# Autodesk Inventor assembly: Assembly
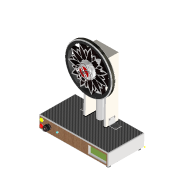
[picture p0: Inventor's stored thumbnail of the model, 180x180]
Saved by Autodesk Inventor 2021 (Build 250183000, 183)
## iProperties
Created: 2021-06-24
Part Number: Assembly
Document SubType Name: Assembly
Designer: RahulRC
Author: RahulRC
## Documents named in this file (10)
- C:\Users\RahulRC\Desktop\Assignments\Exploration\Course_Project\3DModeling\Assembly\Assembly.iam
- C:\Users\RahulRC\Desktop\Assignments\Exploration\Course_Project\3DModeling\Assembly\Design.ipt
- C:\Users\RahulRC\Desktop\Assignments\Exploration\Course_Project\3DModeling\Assembly\DCMotorv2.ipt
- C:\Users\RahulRC\Desktop\Assignments\Exploration\Course_Project\3DModeling\Assembly\rod 2 (1).ipt
- C:\Users\RahulRC\Desktop\Assignments\Exploration\Course_Project\3DModeling\Assembly\buzzer.ipt
- C:\Users\RahulRC\Desktop\Assignments\Exploration\Course_Project\3DModeling\Assembly\base 2.ipt
- C:\Users\RahulRC\Desktop\Assignments\Exploration\Course_Project\3DModeling\Assembly\Attaching Component.ipt
- C:\Users\RahulRC\Desktop\Assignments\Exploration\Course_Project\3DModeling\Assembly\Clamps.ipt
- C:\Users\RahulRC\Desktop\Assignments\Exploration\Course_Project\3DModeling\Assembly\Bolt.ipt
- C:\Users\RahulRC\Desktop\Assignments\Exploration\Course_Project\3DModeling\Assembly\Bolt2.ipt
## Components (17 placed, 9 different names)
1. Design:1 — Mate:1, Mate:2, Angle:1
2. DCMotorv2:1 — Mate:1, Mate:2, Mate:6, Mate:7, Mate:8, Angle:1
3. rod 2 (1):1 — Mate:3, Mate:5
4. buzzer:1 — Mate:4
5. base 2:1 — Mate:3, Mate:4, Mate:9, Mate:10, Mate:21, Mate:22
6. Attaching Component:1 — Mate:5, Mate:6, Mate:7, Mate:8, Mate:31, Mate:32
7. Clamps:1 — Mate:9, Mate:10, Mate:13, Mate:14, Mate:15, Mate:16, Mate:17, Mate:18, Mate:19, Mate:20
8. Bolt:1 — Mate:13, Mate:14
9. Bolt:2 — Mate:17, Mate:19
10. Bolt:3 — Mate:15, Mate:16
11. Bolt:4 — Mate:18, Mate:20
12. Clamps:2 — Mate:21, Mate:22, Mate:23, Mate:24, Mate:25, Mate:26, Mate:27, Mate:28, Mate:29, Mate:30
13. Bolt:5 — Mate:26, Mate:27
14. Bolt:6 — Mate:24, Mate:29
15. Bolt:7 — Mate:25, Mate:28
16. Bolt:8 — Mate:23, Mate:30
17. Bolt2:1 — Mate:31, Mate:32
## Relationships (31: Mate 30, Angle 1)
- Mate:1: Design:1 ↔ DCMotorv2:1
- Mate:2 (2.54 mm): Design:1 ↔ DCMotorv2:1
- Mate:3 (-1 mm): rod 2 (1):1 ↔ base 2:1
- Mate:4: buzzer:1 ↔ base 2:1
- Mate:5: rod 2 (1):1 ↔ Attaching Component:1
- Mate:6: DCMotorv2:1 ↔ Attaching Component:1
- Mate:7: DCMotorv2:1 ↔ Attaching Component:1
- Mate:8: DCMotorv2:1 ↔ Attaching Component:1
- Angle:1 (99640 deg): Design:1 ↔ DCMotorv2:1
- Mate:9: base 2:1 ↔ Clamps:1
- Mate:10: base 2:1 ↔ Clamps:1
- Mate:13: Clamps:1 ↔ Bolt:1
- Mate:14: Clamps:1 ↔ Bolt:1
- Mate:15: Clamps:1 ↔ Bolt:3
- Mate:16: Clamps:1 ↔ Bolt:3
- Mate:17: Clamps:1 ↔ Bolt:2
- Mate:18: Clamps:1 ↔ Bolt:4
- Mate:19: Clamps:1 ↔ Bolt:2
- Mate:20: Clamps:1 ↔ Bolt:4
- Mate:21: base 2:1 ↔ Clamps:2
- Mate:22: base 2:1 ↔ Clamps:2
- Mate:23: Clamps:2 ↔ Bolt:8
- Mate:24: Clamps:2 ↔ Bolt:6
- Mate:25: Clamps:2 ↔ Bolt:7
- Mate:26: Clamps:2 ↔ Bolt:5
- Mate:27: Clamps:2 ↔ Bolt:5
- Mate:28: Clamps:2 ↔ Bolt:7
- Mate:29: Clamps:2 ↔ Bolt:6
- Mate:30: Clamps:2 ↔ Bolt:8
- Mate:31: Attaching Component:1 ↔ Bolt2:1
- Mate:32: Attaching Component:1 ↔ Bolt2:1
